# Autodesk Inventor assembly: Synchronous Belts Transmission
Saved by Autodesk Inventor 2013 (Build 170138000, 138)
## iProperties
Created: 2013-09-18
Part Number: Synchronous Belts Transmission
Document SubType Name: Assembly
Designer: Ian
ClientObjectVersion: 1
Author: Ian
## Documents named in this file (4)
- C:\Users\Ian\Documents\Inventor\xyPartStorage\frame\Design Accelerator\Synchronous Belts Transmission4.iam
- C:\Users\Ian\Documents\Inventor\xyPartStorage\frame\Design Accelerator\Synchronous Belt4.ipt
- C:\Users\Ian\Documents\Inventor\xyPartStorage\frame\Design Accelerator\Synchronous Pulley14.ipt
- C:\Users\Ian\Documents\Inventor\xyPartStorage\frame\Design Accelerator\Synchronous Pulley24.ipt
## Components (3 placed, 3 different names)
1. Synchronous Belt:1 — Flush:1, Mate:1, Mate:2, Flush:2, Mate:3, Mate:4
2. Synchronous Pulley1:1 — Flush:1, Mate:1, Mate:2, Rotation:1
3. Synchronous Pulley2:1 — Flush:2, Mate:3, Rotation:1, Mate:4
## Relationships (7: Mate 4, Flush 2, RelateRotation 1)
- Flush:1: Synchronous Belt:1 ↔ Synchronous Pulley1:1
- Flush:2: Synchronous Belt:1 ↔ Synchronous Pulley2:1
- Rotation:1 [RelateRotation] (2.5 ul): Synchronous Pulley1:1 ↔ Synchronous Pulley2:1
- Mate:1: Synchronous Belt:1 ↔ Synchronous Pulley1:1
- Mate:2: Synchronous Belt:1 ↔ Synchronous Pulley1:1
- Mate:3: Synchronous Belt:1 ↔ Synchronous Pulley2:1
- Mate:4: Synchronous Belt:1 ↔ Synchronous Pulley2:1
